# Autodesk Inventor assembly: GE-12057
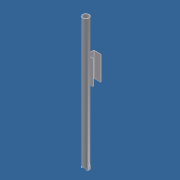
[picture p0: Inventor's stored thumbnail of the model, 180x180]
Saved by Autodesk Inventor 2012 (Build 160160000, 160)
## iProperties
Created: 2011-08-03
Part Number: GE-12057
Document SubType Name: Assembly
Designer: mcyr
Description: Outer Tube, Net Support (left version)
Title: Outer Tube, Net Support (left version)
Author: mcyr
## Documents named in this file (3)
- C:\Data Folder\FRC 2012 Field\Components\GE-12057_left.iam
- C:\Data Folder\FRC 2012 Field\Components\GE-12052_MIR.ipt
- C:\Data Folder\FRC 2012 Field\Components\GE-12057-01_MIR.ipt
## Components (2 placed, 2 different names)
1. GE-12052_MIR:1 — Tangent:3, Tangent:4, Angle:2, Flush:2
2. GE-12057-01_MIR:1 — Tangent:3, Tangent:4, Angle:2, Flush:2
## Relationships (4: Tangent 2, Angle 1, Flush 1)
- Tangent:3 (-41.275 mm): GE-12052_MIR:1 ↔ GE-12057-01_MIR:1
- Tangent:4: GE-12052_MIR:1 ↔ GE-12057-01_MIR:1
- Angle:2 (90 deg): GE-12052_MIR:1 ↔ GE-12057-01_MIR:1
- Flush:2 (228.6 mm): GE-12052_MIR:1 ↔ GE-12057-01_MIR:1
